# Autodesk Inventor assembly: Assembly_Cube_M12_VCAmount_Kinematic_Mirror_90
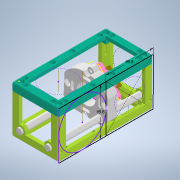
[picture p0: Inventor's stored thumbnail of the model, 180x180]
Saved by Autodesk Inventor 2022 (Build 260153000, 153)
## iProperties
Created: 2022-06-27
Part Number: Assembly_Cube_M12_VCAmount_Kinematic_Mirror_90
Document SubType Name: Assembly
Designer: bingoeleda
Author: bingoeleda
## Documents named in this file (9)
- G:\My Drive\ASP - M.Sc. Photonics\Practical Modules\MODULE 4 - Master Thesis\2.Experiments\Modules\11.Reference_Mirror_Module\Reference_Mirror_with_M12_VCA_Module\Assembly_Cube_M12_VCAmount_Kinematic_Mirror_90.iam
- G:\My Drive\ASP - M.Sc. Photonics\Practical Modules\MODULE 4 - Master Thesis\2.Experiments\Modules\11.Reference_Mirror_Module\Reference_Mirror_with_M12_VCA_Module\20_Cube_Insert_Kinematic_M12_VCAmount_Base_Thorlabs_Cage.ipt
- G:\My Drive\ASP - M.Sc. Photonics\Practical Modules\MODULE 4 - Master Thesis\2.Experiments\Modules\11.Reference_Mirror_Module\Reference_Mirror_with_M12_VCA_Module\20_Cube_Insert_Kinematic_M12_VCAmount__90_pro_v3.ipt
- G:\My Drive\ASP - M.Sc. Photonics\Practical Modules\MODULE 4 - Master Thesis\2.Experiments\Modules\2.Base_Cube\Base_Cube_3DP\Base_Cube_3DP_2x1\with RODS\10_Cube_2x1_v3.ipt
- G:\My Drive\ASP - M.Sc. Photonics\Practical Modules\MODULE 4 - Master Thesis\2.Experiments\Modules\2.Base_Cube\Base_Cube_3DP\Base_Cube_3DP_2x1\with RODS\10_Lid_2x1_v3.ipt
- G:\My Drive\ASP - M.Sc. Photonics\Practical Modules\MODULE 4 - Master Thesis\2.Experiments\Modules\11.Reference_Mirror_Module\Reference_Mirror_with_M12_VCA_Module\00_Thorlabs_Rod_6mm.ipt
- G:\My Drive\ASP - M.Sc. Photonics\Practical Modules\MODULE 4 - Master Thesis\2.Experiments\Modules\11.Reference_Mirror_Module\Reference_Mirror_with_M12_VCA_Module\M12 lens holder.ipt
- G:\My Drive\ASP - M.Sc. Photonics\Practical Modules\MODULE 4 - Master Thesis\2.Experiments\Modules\11.Reference_Mirror_Module\Reference_Mirror_with_M12_VCA_Module\00_coverglass_18mm.ipt
- C:\Users\eda_b\OneDrive\Belgeler\Inventor\Content Center Files\R2022\en-US\DIN 912\DIN 912 - M3 x 0.5 x 6 x 4.75.ipt
## Components (12 placed, 8 different names)
1. 20_Cube_Insert_Kinematic_M12_VCAmount_Base_Thorlabs_Cage:1 — Mate:1, Rotational:2
2. 20_Cube_Insert_Kinematic_M12_VCAmount__90_pro_v3:1 — Rotational:2, Mate:2, Mate:3, Mate:4
3. 10_Cube_2x1_v3:1 — Rotational:1, Rigid:1, Rigid:2, Rotational:3, Rotational:4, Rotational:5, Rotational:6
4. 10_Lid_2x1_v3:1 — Rotational:1
5. 00_Thorlabs_Rod_6mm:1 — Rigid:2, Mate:1
6. 00_Thorlabs_Rod_6mm:2 — Rigid:1
7. M12 lens holder:1 — Mate:2, Mate:3, Mate:4, Rigid:3
8. 00_coverglass_18mm:1 — Rigid:3
9. DIN 912 - replaced by DIN EN ISO 4762 M3 x 6:1 — Rotational:3
10. DIN 912 - replaced by DIN EN ISO 4762 M3 x 6:2 — Rotational:4
11. DIN 912 - replaced by DIN EN ISO 4762 M3 x 6:3 — Rotational:5
12. DIN 912 - replaced by DIN EN ISO 4762 M3 x 6:4 — Rotational:6
## Relationships (13: RevoluteJoint 6, Mate 4, WeldJoint 3)
- Rotational:1 [RevoluteJoint]: 10_Cube_2x1_v3:1 ↔ 10_Lid_2x1_v3:1
- Rigid:1 [WeldJoint] (-2 mm): 10_Cube_2x1_v3:1 ↔ 00_Thorlabs_Rod_6mm:2
- Rigid:2 [WeldJoint] (-2 mm): 10_Cube_2x1_v3:1 ↔ 00_Thorlabs_Rod_6mm:1
- Mate:1: 20_Cube_Insert_Kinematic_M12_VCAmount_Base_Thorlabs_Cage:1 ↔ 00_Thorlabs_Rod_6mm:1
- Rotational:2 [RevoluteJoint]: 20_Cube_Insert_Kinematic_M12_VCAmount_Base_Thorlabs_Cage:1 ↔ 20_Cube_Insert_Kinematic_M12_VCAmount__90_pro_v3:1
- Mate:2: 20_Cube_Insert_Kinematic_M12_VCAmount__90_pro_v3:1 ↔ M12 lens holder:1
- Mate:3: 20_Cube_Insert_Kinematic_M12_VCAmount__90_pro_v3:1 ↔ M12 lens holder:1
- Mate:4: 20_Cube_Insert_Kinematic_M12_VCAmount__90_pro_v3:1 ↔ M12 lens holder:1
- Rigid:3 [WeldJoint]: M12 lens holder:1 ↔ 00_coverglass_18mm:1
- Rotational:3 [RevoluteJoint]: 10_Cube_2x1_v3:1 ↔ DIN 912 - replaced by DIN EN ISO 4762 M3 x 6:1
- Rotational:4 [RevoluteJoint]: 10_Cube_2x1_v3:1 ↔ DIN 912 - replaced by DIN EN ISO 4762 M3 x 6:2
- Rotational:5 [RevoluteJoint]: 10_Cube_2x1_v3:1 ↔ DIN 912 - replaced by DIN EN ISO 4762 M3 x 6:3
- Rotational:6 [RevoluteJoint]: 10_Cube_2x1_v3:1 ↔ DIN 912 - replaced by DIN EN ISO 4762 M3 x 6:4
